# Autodesk Inventor assembly: Socket_CS44_10
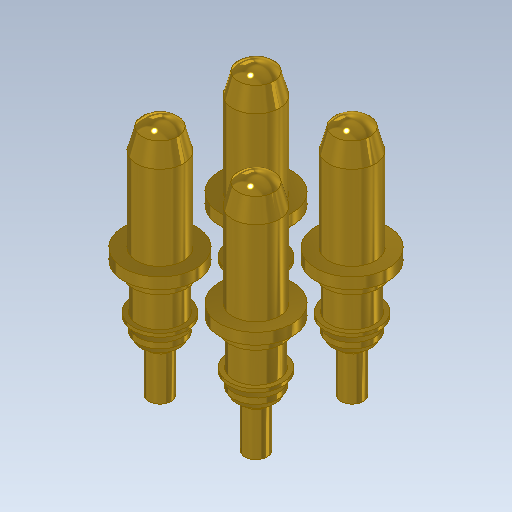
[picture p0: Inventor's stored thumbnail of the model, 512x512]
Saved by Autodesk Inventor 2020 (Build 240168000, 168)
## iProperties
Created: 2013-04-30
Part Number: Socket_CS44_10
Document SubType Name: Assembly
Designer: Mark Neilson
Mass: 0.0279978 g
Surface Area: 0.621371 cm^2
Volume: 0.00808259 cm^3
Density: 3.46397 g/cm^3
Author: Mark Neilson
## Documents named in this file (3)
- C:\Users\alex.lynch\Nextcloud\Documents\UCSD OpenSpeech\CAD\DJB parametric CAD files\200226\Socket_CS44_10.iam
- B:\!!Work\Engineering\Inventor\Vendors\Socket\Knowles\CS44\Socket_CS44_10.ipt
- C:\Users\alex.lynch\Nextcloud\Documents\UCSD OpenSpeech\CAD\DJB parametric CAD files\200226\Socket_Pin_CS.ipt
## Components (5 placed, 2 different names)
1. Socket_CS44_10:1 — Insert:5, Insert:6, Insert:7, Insert:8
2. Socket_Pin_CS:1 — Insert:8
3. Socket_Pin_CS:2 — Insert:7
4. Socket_Pin_CS:3 — Insert:6
5. Socket_Pin_CS:4 — Insert:5
## Relationships (4: Insert 4)
- Insert:5: Socket_CS44_10:1 ↔ Socket_Pin_CS:4
- Insert:6: Socket_CS44_10:1 ↔ Socket_Pin_CS:3
- Insert:7: Socket_CS44_10:1 ↔ Socket_Pin_CS:2
- Insert:8: Socket_CS44_10:1 ↔ Socket_Pin_CS:1
